# Autodesk Inventor assembly: Mecanum Left With Roller 1764
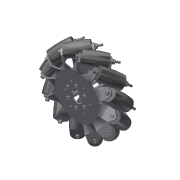
[picture p0: Inventor's stored thumbnail of the model, 180x180]
Saved by Autodesk Inventor 2011 (Build 150239000, 239)
## iProperties
Created: 2011-01-14
Part Number: Mecanum Left With Roller 1764
Document SubType Name: Assembly
Designer: dfranz
Translation Standard: STEP AP203
FileName: //Amserv/amserver/AndyMark/Products/Wheel Mecanum/8 Mecanum Wheel/8 mecanum left with roller.stp
PreProcessor: Unknown
PostProcessor: Build: 239, Release: 2011 RTM - Date: Wed 02/17/2010
Sent Units: millimeter
Uncertainty: 0.001
Author: dfranz
## Documents named in this file (9)
- R:\2010-2011\CMO\Web Site\CADalog\Wheels\Mecanum Wheel 1764\Mecanum Left 1764\Mecanum Left With Roller 1764.iam
- R:\2010-2011\CMO\Web Site\CADalog\Wheels\Mecanum Wheel 1764\Mecanum Left 1764\#10 LockNut 1764.ipt
- R:\2010-2011\CMO\Web Site\CADalog\Wheels\Mecanum Wheel 1764\Mecanum Left 1764\Middle Axle 1764.ipt
- R:\2010-2011\CMO\Web Site\CADalog\Wheels\Mecanum Wheel 1764\Mecanum Left 1764\MBC Bushing MU04TH04 1764.ipt
- R:\2010-2011\CMO\Web Site\CADalog\Wheels\Mecanum Wheel 1764\Mecanum Left 1764\Washer 1764.ipt
- R:\2010-2011\CMO\Web Site\CADalog\Wheels\Mecanum Wheel 1764\Mecanum Left 1764\SHCS 10-32x3_SHCS 10-32x3 1764.ipt
- R:\2010-2011\CMO\Web Site\CADalog\Wheels\Mecanum Wheel 1764\Mecanum Left 1764\Mid Roller III 1764.ipt
- R:\2010-2011\CMO\Web Site\CADalog\Wheels\Mecanum Wheel 1764\Mecanum Left 1764\8 Mecanum Plate Left 1764.ipt
- R:\2010-2011\CMO\Web Site\CADalog\Wheels\Mecanum Wheel 1764\Mecanum Left 1764\Spacer5 1764.ipt
## Components (116 placed, 8 different names)
1. #10 LockNut 1764:1 — Insert:114
2. #10 LockNut 1764:2 — Insert:65
3. #10 LockNut 1764:3 — Insert:42
4. #10 LockNut 1764:4 — Insert:12
5. #10 LockNut 1764:5 — Insert:11
6. #10 LockNut 1764:6 — Insert:82
7. #10 LockNut 1764:7 — Insert:73
8. #10 LockNut 1764:8 — Insert:26
9. #10 LockNut 1764:9 — Insert:9
10. #10 LockNut 1764:10 — Insert:34
11. #10 LockNut 1764:11 — Insert:8
12. #10 LockNut 1764:12 — Insert:105
13. #10 LockNut 1764:13 — Insert:57
14. #10 LockNut 1764:14 — Insert:10
15. #10 LockNut 1764:15 — Insert:49
16. #10 LockNut 1764:16 — Insert:7
17. #10 LockNut 1764:17 — Insert:97
18. #10 LockNut 1764:18 — Insert:90
19. Middle Axle 1764:1 — Insert:52, Insert:53, Insert:55
20. Middle Axle 1764:2 — Insert:68, Insert:69, Insert:70
21. Middle Axle 1764:3 — Insert:96
22. Middle Axle 1764:4 — Insert:36, Insert:37, Insert:39
23. Middle Axle 1764:5 — Insert:84, Insert:85, Insert:87
24. Middle Axle 1764:6 — Insert:28, Insert:29, Insert:30, Insert:31
25. Middle Axle 1764:7 — Insert:100, Insert:101, Insert:103
26. Middle Axle 1764:8 — Insert:108, Insert:109, Insert:111
27. Middle Axle 1764:9 — Insert:44, Insert:45
28. Middle Axle 1764:10 — Insert:21, Insert:22, Insert:24
29. Middle Axle 1764:11 — Insert:76, Insert:77, Insert:79
30. Middle Axle 1764:12 — Insert:60, Insert:61, Insert:62, Insert:63
31. MBC Bushing MU04TH04 1764:1 — Insert:93
32. MBC Bushing MU04TH04 1764:2 — Insert:95
33. MBC Bushing MU04TH04 1764:3 — Insert:56
34. MBC Bushing MU04TH04 1764:4 — Insert:48
35. MBC Bushing MU04TH04 1764:5 — Insert:104
36. MBC Bushing MU04TH04 1764:6 — Insert:64
37. MBC Bushing MU04TH04 1764:7 — Insert:46, Insert:50
38. MBC Bushing MU04TH04 1764:8 — Insert:86
39. MBC Bushing MU04TH04 1764:9 — Insert:30
40. MBC Bushing MU04TH04 1764:10 — Insert:24
41. MBC Bushing MU04TH04 1764:11 — Insert:32
42. MBC Bushing MU04TH04 1764:12 — Insert:110, Insert:113
43. MBC Bushing MU04TH04 1764:13 — Insert:62
44. MBC Bushing MU04TH04 1764:14 — Insert:112
45. MBC Bushing MU04TH04 1764:15 — Insert:80
46. MBC Bushing MU04TH04 1764:16 — Insert:72
47. MBC Bushing MU04TH04 1764:17 — Insert:88
48. MBC Bushing MU04TH04 1764:18 — Insert:38, Insert:41
49. MBC Bushing MU04TH04 1764:19 — Insert:40
50. MBC Bushing MU04TH04 1764:20 — Insert:23
51. MBC Bushing MU04TH04 1764:21 — Insert:78, Insert:81
52. MBC Bushing MU04TH04 1764:22 — Insert:54, Insert:58
53. MBC Bushing MU04TH04 1764:23 — Insert:71, Insert:74
54. MBC Bushing MU04TH04 1764:24 — Insert:102
55. Washer 1764:1 — Insert:53, Insert:54
56. Washer 1764:2 — Insert:92, Insert:93, Insert:98
57. Washer 1764:3 — Insert:70, Insert:72
58. Washer 1764:4 — Insert:85, Insert:86
59. Washer 1764:5 — Insert:22, Insert:23
60. Washer 1764:6 — Insert:109, Insert:110
61. Washer 1764:7 — Insert:94, Insert:95, Insert:96
62. Washer 1764:8 — Insert:31, Insert:32
63. Washer 1764:9 — Insert:61, Insert:66
64. Washer 1764:10 — Insert:103, Insert:104
65. Washer 1764:11 — Insert:63, Insert:64
66. Washer 1764:12 — Insert:37, Insert:38
67. Washer 1764:13 — Insert:79, Insert:80
68. Washer 1764:14 — Insert:39, Insert:40
69. Washer 1764:15 — Insert:20, Insert:21, Insert:25
70. Washer 1764:16 — Insert:77, Insert:78
71. Washer 1764:17 — Insert:29, Insert:33
72. Washer 1764:18 — Insert:55, Insert:56
73. Washer 1764:19 — Insert:111, Insert:112
74. Washer 1764:20 — Insert:101, Insert:102, Insert:106
75. Washer 1764:21 — Insert:45, Insert:46
76. Washer 1764:22 — Insert:87, Insert:88, Insert:89
77. Washer 1764:23 — Insert:69, Insert:71
78. Washer 1764:24 — Insert:47, Insert:48
79. SHCS 10-32x3_SHCS 10-32x3 1764:1 — Insert:3
80. SHCS 10-32x3_SHCS 10-32x3 1764:2 — Insert:99
81. SHCS 10-32x3_SHCS 10-32x3 1764:3 — Insert:43
82. SHCS 10-32x3_SHCS 10-32x3 1764:4 — Insert:19
83. SHCS 10-32x3_SHCS 10-32x3 1764:5 — Insert:5
84. SHCS 10-32x3_SHCS 10-32x3 1764:6 — Insert:4
85. SHCS 10-32x3_SHCS 10-32x3 1764:7 — Insert:59
86. SHCS 10-32x3_SHCS 10-32x3 1764:8 — Insert:35
87. SHCS 10-32x3_SHCS 10-32x3 1764:9 — Insert:107
88. SHCS 10-32x3_SHCS 10-32x3 1764:10 — Insert:91
89. SHCS 10-32x3_SHCS 10-32x3 1764:11 — Insert:2
90. SHCS 10-32x3_SHCS 10-32x3 1764:12 — Insert:67
91. SHCS 10-32x3_SHCS 10-32x3 1764:13 — Insert:83
92. SHCS 10-32x3_SHCS 10-32x3 1764:14 — Insert:1
93. SHCS 10-32x3_SHCS 10-32x3 1764:15 — Insert:75
94. SHCS 10-32x3_SHCS 10-32x3 1764:16 — Insert:27
95. SHCS 10-32x3_SHCS 10-32x3 1764:17 — Insert:51
96. SHCS 10-32x3_SHCS 10-32x3 1764:18 — Insert:6
97. Mid Roller III 1764:1 — Insert:74
98. Mid Roller III 1764:2 — Insert:106
99. Mid Roller III 1764:3 — Insert:25
100. Mid Roller III 1764:4 — Insert:33
101. Mid Roller III 1764:5 — Insert:66
102. Mid Roller III 1764:6 — Insert:113
103. Mid Roller III 1764:7 — Insert:50
104. Mid Roller III 1764:8 — Insert:58
105. Mid Roller III 1764:9 — Insert:81
106. Mid Roller III 1764:10 — Insert:98
107. Mid Roller III 1764:11 — Insert:41
108. Mid Roller III 1764:12 — Insert:89
109. 8 Mecanum Plate Left 1764:1 — Mate:1, Mate:2, Mate:3, Insert:1, Insert:2, Insert:3, Insert:4, Insert:5, Insert:6, Insert:13, Insert:14, Insert:15, Insert:16, Insert:17, Insert:18, Insert:19, Insert:20, Insert:27, Insert:28, Insert:35, Insert:36, Insert:43, Insert:44, Insert:51, Insert:52, Insert:59, Insert:60, Insert:67, Insert:68, Insert:75, Insert:76, Insert:83, Insert:84, Insert:91, Insert:92, Insert:99, Insert:100, Insert:107, Insert:108
110. 8 Mecanum Plate Left 1764:2 — Mate:1, Mate:2, Mate:3, Insert:7, Insert:8, Insert:9, Insert:10, Insert:11, Insert:12, Insert:26, Insert:34, Insert:42, Insert:47, Insert:49, Insert:57, Insert:65, Insert:73, Insert:82, Insert:90, Insert:94, Insert:97, Insert:105, Insert:114
111. Spacer5 1764:1 — Insert:15
112. Spacer5 1764:2 — Insert:13
113. Spacer5 1764:3 — Insert:18
114. Spacer5 1764:4 — Insert:14
115. Spacer5 1764:5 — Insert:16
116. Spacer5 1764:6 — Insert:17
## Relationships (117: Insert 114, Mate 3)
- Mate:1: 8 Mecanum Plate Left 1764:1 ↔ 8 Mecanum Plate Left 1764:2
- Mate:2: 8 Mecanum Plate Left 1764:1 ↔ 8 Mecanum Plate Left 1764:2
- Mate:3 (40.64 mm): 8 Mecanum Plate Left 1764:1 ↔ 8 Mecanum Plate Left 1764:2
- Insert:1: SHCS 10-32x3_SHCS 10-32x3 1764:14 ↔ 8 Mecanum Plate Left 1764:1
- Insert:2: SHCS 10-32x3_SHCS 10-32x3 1764:11 ↔ 8 Mecanum Plate Left 1764:1
- Insert:3: SHCS 10-32x3_SHCS 10-32x3 1764:1 ↔ 8 Mecanum Plate Left 1764:1
- Insert:4: SHCS 10-32x3_SHCS 10-32x3 1764:6 ↔ 8 Mecanum Plate Left 1764:1
- Insert:5: SHCS 10-32x3_SHCS 10-32x3 1764:5 ↔ 8 Mecanum Plate Left 1764:1
- Insert:6: SHCS 10-32x3_SHCS 10-32x3 1764:18 ↔ 8 Mecanum Plate Left 1764:1
- Insert:7: #10 LockNut 1764:16 ↔ 8 Mecanum Plate Left 1764:2
- Insert:8: #10 LockNut 1764:11 ↔ 8 Mecanum Plate Left 1764:2
- Insert:9: #10 LockNut 1764:9 ↔ 8 Mecanum Plate Left 1764:2
- Insert:10: #10 LockNut 1764:14 ↔ 8 Mecanum Plate Left 1764:2
- Insert:11: #10 LockNut 1764:5 ↔ 8 Mecanum Plate Left 1764:2
- Insert:12: #10 LockNut 1764:4 ↔ 8 Mecanum Plate Left 1764:2
- Insert:13: 8 Mecanum Plate Left 1764:1 ↔ Spacer5 1764:2
- Insert:14: 8 Mecanum Plate Left 1764:1 ↔ Spacer5 1764:4
- Insert:15: 8 Mecanum Plate Left 1764:1 ↔ Spacer5 1764:1
- Insert:16: 8 Mecanum Plate Left 1764:1 ↔ Spacer5 1764:5
- Insert:17: 8 Mecanum Plate Left 1764:1 ↔ Spacer5 1764:6
- Insert:18: 8 Mecanum Plate Left 1764:1 ↔ Spacer5 1764:3
- Insert:19: SHCS 10-32x3_SHCS 10-32x3 1764:4 ↔ 8 Mecanum Plate Left 1764:1
- Insert:20: Washer 1764:15 ↔ 8 Mecanum Plate Left 1764:1
- Insert:21: Middle Axle 1764:10 ↔ Washer 1764:15
- Insert:22: Middle Axle 1764:10 ↔ Washer 1764:5
- Insert:23: MBC Bushing MU04TH04 1764:20 ↔ Washer 1764:5
- Insert:24: Middle Axle 1764:10 ↔ MBC Bushing MU04TH04 1764:10
- Insert:25: Washer 1764:15 ↔ Mid Roller III 1764:3
- Insert:26: #10 LockNut 1764:8 ↔ 8 Mecanum Plate Left 1764:2
- Insert:27: SHCS 10-32x3_SHCS 10-32x3 1764:16 ↔ 8 Mecanum Plate Left 1764:1
- Insert:28: Middle Axle 1764:6 ↔ 8 Mecanum Plate Left 1764:1
- Insert:29: Middle Axle 1764:6 ↔ Washer 1764:17
- Insert:30: Middle Axle 1764:6 ↔ MBC Bushing MU04TH04 1764:9
- Insert:31: Middle Axle 1764:6 ↔ Washer 1764:8
- Insert:32: MBC Bushing MU04TH04 1764:11 ↔ Washer 1764:8
- Insert:33: Washer 1764:17 ↔ Mid Roller III 1764:4
- Insert:34: #10 LockNut 1764:10 ↔ 8 Mecanum Plate Left 1764:2
- Insert:35: SHCS 10-32x3_SHCS 10-32x3 1764:8 ↔ 8 Mecanum Plate Left 1764:1
- Insert:36: Middle Axle 1764:4 ↔ 8 Mecanum Plate Left 1764:1
- Insert:37: Middle Axle 1764:4 ↔ Washer 1764:12
- Insert:38: MBC Bushing MU04TH04 1764:18 ↔ Washer 1764:12
- Insert:39: Middle Axle 1764:4 ↔ Washer 1764:14
- Insert:40: MBC Bushing MU04TH04 1764:19 ↔ Washer 1764:14
- Insert:41: MBC Bushing MU04TH04 1764:18 ↔ Mid Roller III 1764:11
- Insert:42: #10 LockNut 1764:3 ↔ 8 Mecanum Plate Left 1764:2
- Insert:43: SHCS 10-32x3_SHCS 10-32x3 1764:3 ↔ 8 Mecanum Plate Left 1764:1
- Insert:44: Middle Axle 1764:9 ↔ 8 Mecanum Plate Left 1764:1
- Insert:45: Middle Axle 1764:9 ↔ Washer 1764:21
- Insert:46: MBC Bushing MU04TH04 1764:7 ↔ Washer 1764:21
- Insert:47: Washer 1764:24 ↔ 8 Mecanum Plate Left 1764:2
- Insert:48: MBC Bushing MU04TH04 1764:4 ↔ Washer 1764:24
- Insert:49: #10 LockNut 1764:15 ↔ 8 Mecanum Plate Left 1764:2
- Insert:50: MBC Bushing MU04TH04 1764:7 ↔ Mid Roller III 1764:7
- Insert:51: SHCS 10-32x3_SHCS 10-32x3 1764:17 ↔ 8 Mecanum Plate Left 1764:1
- Insert:52: Middle Axle 1764:1 ↔ 8 Mecanum Plate Left 1764:1
- Insert:53: Middle Axle 1764:1 ↔ Washer 1764:1
- Insert:54: MBC Bushing MU04TH04 1764:22 ↔ Washer 1764:1
- Insert:55: Middle Axle 1764:1 ↔ Washer 1764:18
- Insert:56: MBC Bushing MU04TH04 1764:3 ↔ Washer 1764:18
- Insert:57: #10 LockNut 1764:13 ↔ 8 Mecanum Plate Left 1764:2
- Insert:58: MBC Bushing MU04TH04 1764:22 ↔ Mid Roller III 1764:8
- Insert:59: SHCS 10-32x3_SHCS 10-32x3 1764:7 ↔ 8 Mecanum Plate Left 1764:1
- Insert:60: Middle Axle 1764:12 ↔ 8 Mecanum Plate Left 1764:1
- Insert:61: Middle Axle 1764:12 ↔ Washer 1764:9
- Insert:62: Middle Axle 1764:12 ↔ MBC Bushing MU04TH04 1764:13
- Insert:63: Middle Axle 1764:12 ↔ Washer 1764:11
- Insert:64: MBC Bushing MU04TH04 1764:6 ↔ Washer 1764:11
- Insert:65: #10 LockNut 1764:2 ↔ 8 Mecanum Plate Left 1764:2
- Insert:66: Washer 1764:9 ↔ Mid Roller III 1764:5
- Insert:67: SHCS 10-32x3_SHCS 10-32x3 1764:12 ↔ 8 Mecanum Plate Left 1764:1
- Insert:68: Middle Axle 1764:2 ↔ 8 Mecanum Plate Left 1764:1
- Insert:69: Middle Axle 1764:2 ↔ Washer 1764:23
- Insert:70: Middle Axle 1764:2 ↔ Washer 1764:3
- Insert:71: MBC Bushing MU04TH04 1764:23 ↔ Washer 1764:23
- Insert:72: MBC Bushing MU04TH04 1764:16 ↔ Washer 1764:3
- Insert:73: #10 LockNut 1764:7 ↔ 8 Mecanum Plate Left 1764:2
- Insert:74: MBC Bushing MU04TH04 1764:23 ↔ Mid Roller III 1764:1
- Insert:75: SHCS 10-32x3_SHCS 10-32x3 1764:15 ↔ 8 Mecanum Plate Left 1764:1
- Insert:76: Middle Axle 1764:11 ↔ 8 Mecanum Plate Left 1764:1
- Insert:77: Middle Axle 1764:11 ↔ Washer 1764:16
- Insert:78: MBC Bushing MU04TH04 1764:21 ↔ Washer 1764:16
- Insert:79: Middle Axle 1764:11 ↔ Washer 1764:13
- Insert:80: MBC Bushing MU04TH04 1764:15 ↔ Washer 1764:13
- Insert:81: MBC Bushing MU04TH04 1764:21 ↔ Mid Roller III 1764:9
- Insert:82: #10 LockNut 1764:6 ↔ 8 Mecanum Plate Left 1764:2
- Insert:83: SHCS 10-32x3_SHCS 10-32x3 1764:13 ↔ 8 Mecanum Plate Left 1764:1
- Insert:84: Middle Axle 1764:5 ↔ 8 Mecanum Plate Left 1764:1
- Insert:85: Middle Axle 1764:5 ↔ Washer 1764:4
- Insert:86: MBC Bushing MU04TH04 1764:8 ↔ Washer 1764:4
- Insert:87: Middle Axle 1764:5 ↔ Washer 1764:22
- Insert:88: MBC Bushing MU04TH04 1764:17 ↔ Washer 1764:22
- Insert:89: Washer 1764:22 ↔ Mid Roller III 1764:12
- Insert:90: #10 LockNut 1764:18 ↔ 8 Mecanum Plate Left 1764:2
- Insert:91: SHCS 10-32x3_SHCS 10-32x3 1764:10 ↔ 8 Mecanum Plate Left 1764:1
- Insert:92: Washer 1764:2 ↔ 8 Mecanum Plate Left 1764:1
- Insert:93: MBC Bushing MU04TH04 1764:1 ↔ Washer 1764:2
- Insert:94: Washer 1764:7 ↔ 8 Mecanum Plate Left 1764:2
- Insert:95: MBC Bushing MU04TH04 1764:2 ↔ Washer 1764:7
- Insert:96: Middle Axle 1764:3 ↔ Washer 1764:7
- Insert:97: #10 LockNut 1764:17 ↔ 8 Mecanum Plate Left 1764:2
- Insert:98: Washer 1764:2 ↔ Mid Roller III 1764:10
- Insert:99: SHCS 10-32x3_SHCS 10-32x3 1764:2 ↔ 8 Mecanum Plate Left 1764:1
- Insert:100: Middle Axle 1764:7 ↔ 8 Mecanum Plate Left 1764:1
- Insert:101: Middle Axle 1764:7 ↔ Washer 1764:20
- Insert:102: MBC Bushing MU04TH04 1764:24 ↔ Washer 1764:20
- Insert:103: Middle Axle 1764:7 ↔ Washer 1764:10
- Insert:104: MBC Bushing MU04TH04 1764:5 ↔ Washer 1764:10
- Insert:105: #10 LockNut 1764:12 ↔ 8 Mecanum Plate Left 1764:2
- Insert:106: Washer 1764:20 ↔ Mid Roller III 1764:2
- Insert:107: SHCS 10-32x3_SHCS 10-32x3 1764:9 ↔ 8 Mecanum Plate Left 1764:1
- Insert:108: Middle Axle 1764:8 ↔ 8 Mecanum Plate Left 1764:1
- Insert:109: Middle Axle 1764:8 ↔ Washer 1764:6
- Insert:110: MBC Bushing MU04TH04 1764:12 ↔ Washer 1764:6
- Insert:111: Middle Axle 1764:8 ↔ Washer 1764:19
- Insert:112: MBC Bushing MU04TH04 1764:14 ↔ Washer 1764:19
- Insert:113: MBC Bushing MU04TH04 1764:12 ↔ Mid Roller III 1764:6
- Insert:114: #10 LockNut 1764:1 ↔ 8 Mecanum Plate Left 1764:2
